# Autodesk Inventor assembly: Walls
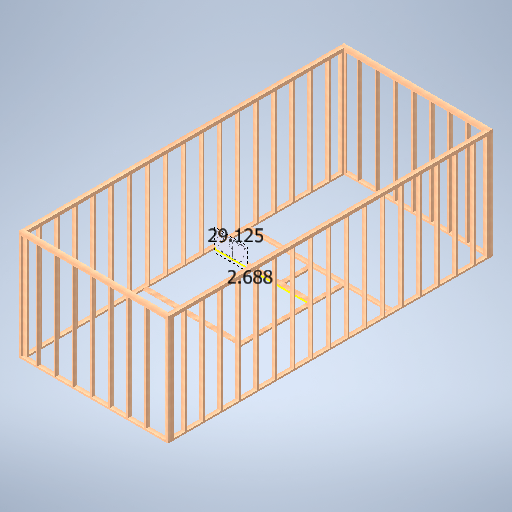
[picture p0: Inventor's stored thumbnail of the model, 512x512]
Saved by Autodesk Inventor 2025.1 (Build 291241020, 241B)
## iProperties
Created: 2024-09-15
Part Number: Walls
Document SubType Name: Assembly
Designer: Tom
Author: Tom
## Documents named in this file (11)
- C:\Users\Tom\Documents\Inventor\Mobility\Additional_Building\Walls.iam
- C:\Users\Tom\Documents\Inventor\Mobility\Additional_Building\Plate_With_Length_144_Inches.ipt
- C:\Users\Tom\Documents\Inventor\Mobility\Additional_Building\Plate_With_Length_125_Inches.ipt
- C:\Users\Tom\Documents\Inventor\Mobility\Additional_Building\California_Corner.iam
- C:\Users\Tom\Documents\Inventor\Mobility\Additional_Building\Stud_With_Height_93_Inches.ipt
- C:\Users\Tom\Documents\Inventor\Mobility\Additional_Building\Plate_With_Length_132_Inches.ipt
- C:\Users\Tom\Documents\Inventor\Mobility\Additional_Building\Plate_With_Length_68.5_Inches.ipt
- C:\Users\Tom\Documents\Inventor\Mobility\Additional_Building\Plate_With_Length_86.5625_Inches_And_Image_Of_Bath_Tub.ipt
- C:\Users\Tom\Documents\Inventor\Mobility\Additional_Building\Plate_With_Length_60_Inches.ipt
- C:\Users\Tom\Documents\Inventor\Mobility\Additional_Building\Plate_With_Length_25_Inches.ipt
- C:\Users\Tom\Documents\Inventor\Mobility\Additional_Building\Plate_With_Length_86.5625_Inches.ipt
## Components (78 placed, 10 different names)
1. California_Corner:1 [sub-assembly] — Mate:2, Flush:3, Flush:4
2. California_Corner:2 [sub-assembly] — Mate:13, Flush:13, Flush:14, Flush:19, Flush:20, Flush:21
3. California_Corner:3 [sub-assembly] — Mate:14, Flush:15, Flush:16
4. California_Corner:4 [sub-assembly] — Mate:15, Flush:17, Flush:18
5. Plate_With_Length_125_Inches:5 — Mate:16, Flush:22, Mate:17, Mate:19, Mate:24, Flush:27
6. Plate_With_Length_60_Inches:1 — Mate:19, Mate:27, Mate:31
7. Plate_With_Length_25_Inches:1 — Mate:25, Mate:28
8. Plate_With_Length_25_Inches:2 — Mate:24, Flush:27, Mate:25, Mate:29
9. Plate_With_Length_86.5625_Inches_And_Image_Of_Bath_Tub:1 — Mate:26, Flush:28, Mate:27, Mate:28, Mate:29
10. Plate_With_Length_86.5625_Inches:1 — Mate:30, Mate:31, Flush:29
11. Plate_With_Length_132_Inches:1 — Mate:8, Flush:9, Flush:10, Mate:10
12. Plate_With_Length_132_Inches:2
13. Plate_With_Length_144_Inches:9 — Mate:11, Mate:12, Flush:12
14. Plate_With_Length_144_Inches:10
15. Plate_With_Length_144_Inches:1 — Flush:5, Mate:15, Flush:17, Flush:18, Mate:30, Flush:29
16. Plate_With_Length_144_Inches:2 — Mate:14, Flush:15, Flush:16, Mate:26, Flush:28
17. Plate_With_Length_144_Inches:3 — Mate:1, Flush:1, Flush:2, Mate:4, Flush:6, Mate:13, Flush:13, Flush:14, Mate:16, Flush:22
18. Plate_With_Length_144_Inches:4 — Mate:2, Flush:3, Flush:4
19. Plate_With_Length_125_Inches:1 — Mate:1, Flush:1, Flush:2, Mate:3, Mate:7
20. Plate_With_Length_125_Inches:2 — Mate:17
21. Plate_With_Length_144_Inches:5 — Flush:9
22. Plate_With_Length_144_Inches:6
23. Plate_With_Length_144_Inches:7 — Mate:9, Flush:11
24. Plate_With_Length_144_Inches:8 — Mate:11, Flush:12
25. Plate_With_Length_125_Inches:3 — Flush:7, Mate:8, Flush:10
26. Plate_With_Length_125_Inches:4
27. Stud_With_Height_93_Inches:1 — Mate:4, Flush:6, Flush:19
28. Stud_With_Height_93_Inches:2
29. Stud_With_Height_93_Inches:3
30. Stud_With_Height_93_Inches:4
31. Stud_With_Height_93_Inches:5
32. Stud_With_Height_93_Inches:6
33. Stud_With_Height_93_Inches:7
34. Stud_With_Height_93_Inches:8
35. Stud_With_Height_93_Inches:9
36. Stud_With_Height_93_Inches:10
37. Stud_With_Height_93_Inches:11
38. Stud_With_Height_93_Inches:33
39. Stud_With_Height_93_Inches:34
40. Stud_With_Height_93_Inches:35
41. Stud_With_Height_93_Inches:36
42. Stud_With_Height_93_Inches:37
43. Stud_With_Height_93_Inches:38
44. Stud_With_Height_93_Inches:12
45. Stud_With_Height_93_Inches:13
46. Stud_With_Height_93_Inches:14
47. Stud_With_Height_93_Inches:15
48. Stud_With_Height_93_Inches:16
49. Stud_With_Height_93_Inches:17
50. Stud_With_Height_93_Inches:18
51. Stud_With_Height_93_Inches:19
52. Stud_With_Height_93_Inches:20
53. Stud_With_Height_93_Inches:21
54. Stud_With_Height_93_Inches:22
55. Stud_With_Height_93_Inches:39
56. Stud_With_Height_93_Inches:40
57. Stud_With_Height_93_Inches:41
58. Stud_With_Height_93_Inches:42
59. Stud_With_Height_93_Inches:43
60. Stud_With_Height_93_Inches:44
61. Stud_With_Height_93_Inches:23 — Flush:7, Mate:7, Flush:20
62. Stud_With_Height_93_Inches:24
63. Stud_With_Height_93_Inches:25
64. Stud_With_Height_93_Inches:26
65. Stud_With_Height_93_Inches:27
66. Stud_With_Height_93_Inches:45
67. Stud_With_Height_93_Inches:46
68. Stud_With_Height_93_Inches:28
69. Stud_With_Height_93_Inches:29
70. Stud_With_Height_93_Inches:30
71. Stud_With_Height_93_Inches:31
72. Stud_With_Height_93_Inches:32
73. Stud_With_Height_93_Inches:47
74. Stud_With_Height_93_Inches:48
75. Plate_With_Length_68.5_Inches:1 — Mate:9, Mate:10, Flush:11
76. Plate_With_Length_68.5_Inches:2 — Mate:12
77. Plate_With_Length_68.5_Inches:3
78. Plate_With_Length_68.5_Inches:4
## Component patterns: (2 elements), (2 elements), (2 elements), (2 elements, first: Plate_With_Length_132_Inches:1), (2 elements, first: Plate_With_Length_144_Inches:9), (4 elements, first: Plate_With_Length_144_Inches:1), (2 elements, first: Plate_With_Length_125_Inches:1), Component Pattern 1:2 (4 elements), Component Pattern 2:2 (2 elements), (17 elements, first: Stud_With_Height_93_Inches:1), Component Pattern 4:2 (17 elements), (7 elements, first: Stud_With_Height_93_Inches:23), Component Pattern 6:2 (7 elements), (2 elements, first: Plate_With_Length_68.5_Inches:1), Component Pattern 10:2 (2 elements)
## Relationships (48: Mate 24, Flush 24)
- Mate:1: Plate_With_Length_144_Inches:3 ↔ Plate_With_Length_125_Inches:1
- Flush:1: Plate_With_Length_144_Inches:3 ↔ Plate_With_Length_125_Inches:1
- Flush:2: Plate_With_Length_144_Inches:3 ↔ Plate_With_Length_125_Inches:1
- Mate:2: California_Corner:1 ↔ Plate_With_Length_144_Inches:4
- Flush:3: California_Corner:1 ↔ Plate_With_Length_144_Inches:4
- Flush:4: California_Corner:1 ↔ Plate_With_Length_144_Inches:4
- Flush:5: Plate_With_Length_144_Inches:1
- Mate:3 (1536.7 mm): Plate_With_Length_125_Inches:1
- Mate:4: Plate_With_Length_144_Inches:3 ↔ Stud_With_Height_93_Inches:1
- Flush:6: Plate_With_Length_144_Inches:3 ↔ Stud_With_Height_93_Inches:1
- Flush:7: Plate_With_Length_125_Inches:3 ↔ Stud_With_Height_93_Inches:23
- Mate:7: Plate_With_Length_125_Inches:1 ↔ Stud_With_Height_93_Inches:23
- Mate:8: Plate_With_Length_132_Inches:1 ↔ Plate_With_Length_125_Inches:3
- Flush:9: Plate_With_Length_132_Inches:1 ↔ Plate_With_Length_144_Inches:5
- Flush:10: Plate_With_Length_132_Inches:1 ↔ Plate_With_Length_125_Inches:3
- Mate:9: Plate_With_Length_144_Inches:7 ↔ Plate_With_Length_68.5_Inches:1
- Mate:10: Plate_With_Length_132_Inches:1 ↔ Plate_With_Length_68.5_Inches:1
- Flush:11: Plate_With_Length_144_Inches:7 ↔ Plate_With_Length_68.5_Inches:1
- Mate:11: Plate_With_Length_144_Inches:9 ↔ Plate_With_Length_144_Inches:8
- Mate:12: Plate_With_Length_144_Inches:9 ↔ Plate_With_Length_68.5_Inches:2
- Flush:12: Plate_With_Length_144_Inches:9 ↔ Plate_With_Length_144_Inches:8
- Mate:13: California_Corner:2 ↔ Plate_With_Length_144_Inches:3
- Flush:13: California_Corner:2 ↔ Plate_With_Length_144_Inches:3
- Flush:14: California_Corner:2 ↔ Plate_With_Length_144_Inches:3
- Mate:14: California_Corner:3 ↔ Plate_With_Length_144_Inches:2
- Flush:15: California_Corner:3 ↔ Plate_With_Length_144_Inches:2
- Flush:16: California_Corner:3 ↔ Plate_With_Length_144_Inches:2
- Mate:15: California_Corner:4 ↔ Plate_With_Length_144_Inches:1
- Flush:17: California_Corner:4 ↔ Plate_With_Length_144_Inches:1
- Flush:18: California_Corner:4 ↔ Plate_With_Length_144_Inches:1
- Flush:19 (387.35 mm): California_Corner:2 ↔ Stud_With_Height_93_Inches:1
- Flush:20 (501.65 mm): California_Corner:2 ↔ Stud_With_Height_93_Inches:23
- Flush:21 (15.875 mm): California_Corner:2
- Mate:16: Plate_With_Length_125_Inches:5 ↔ Plate_With_Length_144_Inches:3
- Flush:22: Plate_With_Length_125_Inches:5 ↔ Plate_With_Length_144_Inches:3
- Mate:17 (2092.325 mm): Plate_With_Length_125_Inches:5 ↔ Plate_With_Length_125_Inches:2
- Mate:19 (723.9 mm): Plate_With_Length_125_Inches:5 ↔ Plate_With_Length_60_Inches:1
- Mate:24: Plate_With_Length_125_Inches:5 ↔ Plate_With_Length_25_Inches:2
- Flush:27: Plate_With_Length_125_Inches:5 ↔ Plate_With_Length_25_Inches:2
- Mate:25 (635 mm): Plate_With_Length_25_Inches:1 ↔ Plate_With_Length_25_Inches:2
- Mate:26: Plate_With_Length_86.5625_Inches_And_Image_Of_Bath_Tub:1 ↔ Plate_With_Length_144_Inches:2
- Flush:28: Plate_With_Length_86.5625_Inches_And_Image_Of_Bath_Tub:1 ↔ Plate_With_Length_144_Inches:2
- Mate:27: Plate_With_Length_60_Inches:1 ↔ Plate_With_Length_86.5625_Inches_And_Image_Of_Bath_Tub:1
- Mate:28: Plate_With_Length_25_Inches:1 ↔ Plate_With_Length_86.5625_Inches_And_Image_Of_Bath_Tub:1
- Mate:29: Plate_With_Length_25_Inches:2 ↔ Plate_With_Length_86.5625_Inches_And_Image_Of_Bath_Tub:1
- Mate:30: Plate_With_Length_86.5625_Inches:1 ↔ Plate_With_Length_144_Inches:1
- Mate:31: Plate_With_Length_60_Inches:1 ↔ Plate_With_Length_86.5625_Inches:1
- Flush:29: Plate_With_Length_86.5625_Inches:1 ↔ Plate_With_Length_144_Inches:1
